# Autodesk Inventor assembly: NRF24l01_with_antenna
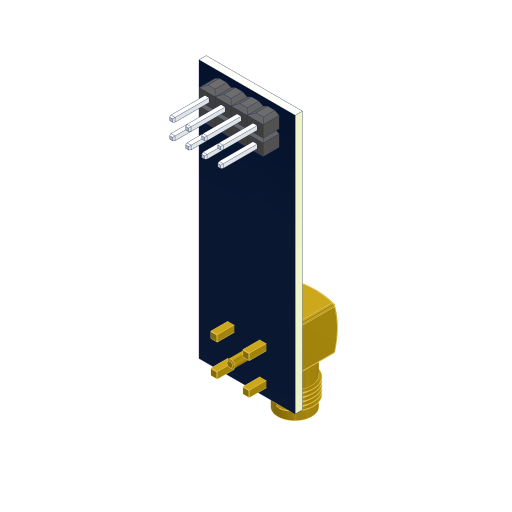
[picture p0: Inventor's stored thumbnail of the model, 512x512]
Saved by Autodesk Inventor 2023.1 (Build 271208000, 208)
## iProperties
Created: 2017-12-17
Part Number: NRF24l01_with_antenna
Description: STEP AP214
Document SubType Name: Assembly
Designer: tland
Sending System: SolidWorks 2017
Preprocessor: SwSTEP 2.0
Title: NRF24l01_with_antenna.STEP
Revision Number: ANY
## Documents named in this file (6)
- D:\FH-Studium\Master\Masterarbeit\Masterarbeit\CAD\components\nrf24l01-pa-lna\NRF24l01_without_antenna.iam
- D:\FH-Studium\Master\Masterarbeit\Masterarbeit\CAD\components\nrf24l01-pa-lna\NRF24L01_PCB.ipt
- D:\FH-Studium\Master\Masterarbeit\Masterarbeit\CAD\components\nrf24l01-pa-lna\male header.ipt
- D:\FH-Studium\Master\Masterarbeit\Masterarbeit\CAD\components\nrf24l01-pa-lna\NRF24L01_SMA-angled.ipt
- D:\FH-Studium\Master\Masterarbeit\Masterarbeit\CAD\components\nrf24l01-pa-lna\NRF24L01-CHIP-NRF___ _________.ipt
- D:\FH-Studium\Master\Masterarbeit\Masterarbeit\CAD\components\nrf24l01-pa-lna\User Library-QFN-16_3x3.iam
## Components (12 placed, 12 different names)
1. NRF24L01_PCB_1 — Symmetrie:1
2. male header_2
3. male header_3
4. male header_4
5. male header_5
6. male header_6
7. male header_7
8. male header_8
9. male header_9
10. NRF24L01_SMA-angled_10
11. NRF24L01-CHIP-NRF___ __________11
12. User Library-QFN-16_3x3_12 [sub-assembly]
## Relationships (1: Symmetry 1)
- Symmetrie:1: NRF24L01_PCB_1
